# Autodesk Inventor assembly: kladka
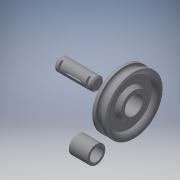
[picture p0: Inventor's stored thumbnail of the model, 180x180]
Saved by Autodesk Inventor 2019 (Build 230136000, 136)
## iProperties
Created: 2018-11-24
Part Number: kladka
Document SubType Name: Assembly
Designer: Radek
Author: Radek
## Documents named in this file (4)
- C:\Users\MJ\Documents\AiFit-Inventor\Resources\kladka\kladka.iam
- C:\Users\MJ\Documents\AiFit-Inventor\Resources\kladka\pouzdro.ipt
- C:\Users\MJ\Documents\AiFit-Inventor\Resources\kladka\čep.ipt
- C:\Users\MJ\Documents\AiFit-Inventor\Resources\kladka\kladka.ipt
## Components (3 placed, 3 different names)
1. pouzdro:1
2. čep:1 — Proti sobě:1
3. kladka:1 — Proti sobě:1
## Relationships (1: Mate 1)
- Proti sobě:1 [Mate]: čep:1 ↔ kladka:1
